# Autodesk Inventor assembly: Assembly2
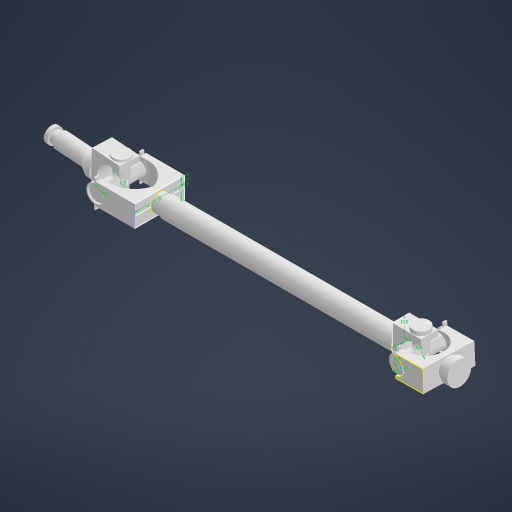
[picture p0: Inventor's stored thumbnail of the model, 512x512]
Saved by Autodesk Inventor 2023 (Build 270158030, 158C)
## iProperties
Created: 2023-02-03
Part Number: Assembly2
Document SubType Name: Assembly
Designer: Monster
Author: Monster
## Documents named in this file (6)
- C:\Users\Monster\Desktop\Ders\UKA\shaft\Assembly2.iam
- C:\Users\Monster\Desktop\Ders\UKA\shaft\Part1.ipt
- C:\Users\Monster\Desktop\Ders\UKA\shaft\Part2.ipt
- C:\Users\Monster\Desktop\Ders\UKA\shaft\Part4.ipt
- C:\Users\Monster\Desktop\Ders\UKA\shaft\Part5.ipt
- C:\Users\Monster\Desktop\Ders\UKA\shaft\Part3.ipt
## Components (9 placed, 5 different names)
1. Part1:1 — Mate:1, Mate:2, Mate:3, Mate:4, Mate:9, Mate:11
2. Part2:1 — Mate:1, Mate:2, Mate:6, Mate:7, Mate:12, Mate:14
3. Part2:2 — Mate:3, Mate:4, Mate:5, Flush:1, Mate:8, Mate:10
4. Part4:1 — Mate:5, Flush:1
5. Part5:1 — Mate:6, Mate:7, Mate:13, Mate:15
6. Part3:1 — Mate:8, Mate:9
7. Part3:2 — Mate:10, Mate:11
8. Part3:3 — Mate:12, Mate:13
9. Part3:4 — Mate:14, Mate:15
## Relationships (16: Mate 15, Flush 1)
- Mate:1: Part1:1 ↔ Part2:1
- Mate:2: Part1:1 ↔ Part2:1
- Mate:3: Part1:1 ↔ Part2:2
- Mate:4 (1 mm): Part1:1 ↔ Part2:2
- Mate:5: Part2:2 ↔ Part4:1
- Flush:1 (1 mm): Part2:2 ↔ Part4:1
- Mate:6: Part2:1 ↔ Part5:1
- Mate:7: Part2:1 ↔ Part5:1
- Mate:8: Part2:2 ↔ Part3:1
- Mate:9: Part1:1 ↔ Part3:1
- Mate:10: Part2:2 ↔ Part3:2
- Mate:11: Part1:1 ↔ Part3:2
- Mate:12: Part2:1 ↔ Part3:3
- Mate:13: Part5:1 ↔ Part3:3
- Mate:14: Part2:1 ↔ Part3:4
- Mate:15: Part5:1 ↔ Part3:4
